# Autodesk Inventor assembly: tip_3_n_base_ass
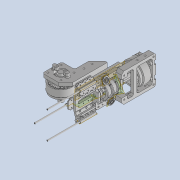
[picture p0: Inventor's stored thumbnail of the model, 180x180]
Saved by Autodesk Inventor 2020 (Build 240168000, 168)
## iProperties
Created: 2021-10-06
Part Number: tip_3_n_base_ass
Document SubType Name: Assembly
Designer: Shuang Peng
Author: Shuang Peng
## Documents named in this file (14)
- D:\projects-3\torque fb tip\hardware\tip_3\tip_3_n_base_ass.iam
- D:\projects-3\torque fb tip\hardware\tip_3\roller_n_1.ipt
- D:\projects-3\torque fb tip\hardware\tip_3\bearing_hh_1.ipt
- D:\projects-3\torque fb tip\hardware\tip_3\bearing_3_6_2.ipt
- D:\projects-3\torque fb tip\hardware\tip_3\pin3_40.ipt
- D:\projects-3\torque fb tip\hardware\tip_3\end_shell_n_1.ipt
- D:\projects-3\torque fb tip\hardware\tip_3\c_roller_1.ipt
- D:\projects-3\torque fb tip\hardware\tip_3\bl_tube_ass_2.iam
- D:\projects-3\torque fb tip\hardware\tip_3\ext_pin_shell_2.ipt
- D:\projects-3\torque fb tip\hardware\tip_3\mot_test_enc_hh_1.ipt
- D:\projects-3\torque fb tip\hardware\tip_3\mot_27_ass.iam
- D:\projects-3\torque fb tip\hardware\tip_3\mot_trans_1.ipt
- D:\projects-3\torque fb tip\hardware\tip_3\arc_wheel_shell_1.ipt
- D:\projects-3\torque fb tip\hardware\tip_3\tendon_wh_1_mod.ipt
## Components (24 placed, 13 different names)
1. roller_n_1:1 — Insert:1, Insert:2, Insert:5
2. roller_n_1:2 — Insert:1, Insert:2, Insert:6, Flush:3
3. bearing_hh_1:1 — Insert:3, Flush:1, Flush:2
4. bearing_hh_1:2 — Insert:4, Flush:1, Insert:8
5. bearing_3_6_2:1 — Insert:4, Insert:6
6. bearing_3_6_2:2 — Insert:3, Insert:5, Insert:7
7. pin3_40:1 — Insert:7
8. end_shell_n_1:1 — Flush:2, Insert:8, Flush:3, Insert:10, Insert:12, Flush:4, Mate:1, Flush:5, Insert:17
9. c_roller_1:1 — Insert:9
10. bearing_3_6_2:3 — Insert:9, Insert:10
11. c_roller_1:2
12. bearing_3_6_2:4 — Insert:12
13. bl_tube_ass_2:1 [sub-assembly] — Insert:22, Insert:23
14. bl_tube_ass_2:2 [sub-assembly] — Insert:20, Insert:21
15. bl_tube_ass_2:3 [sub-assembly] — Insert:18, Insert:19
16. ext_pin_shell_2:1 — Flush:4, Mate:1, Flush:5, Angle:1, Insert:18, Insert:19, Insert:20, Insert:21, Insert:22, Insert:23, Flush:6, Insert:24, Insert:25
17. mot_test_enc_hh_1:1 — Insert:13, Insert:14, Angle:1
18. mot_27_ass:1 [sub-assembly] — Insert:13, Insert:14, Insert:15, Insert:16
19. mot_trans_1:1 — Insert:15, Insert:16, Insert:17
20. arc_wheel_shell_1:1 — Flush:6, Insert:24, Insert:25, Insert:27, Flush:7
21. c_roller_1:3
22. bearing_3_6_2:5 — Insert:27
23. mot_27_ass:2 [sub-assembly] — Flush:7, Insert:28, Insert:29
24. tendon_wh_1_mod:1 — Insert:28, Insert:29
## Relationships (38: Insert 29, Flush 7, Mate 1, Angle 1)
- Insert:1: roller_n_1:1 ↔ roller_n_1:2
- Insert:2: roller_n_1:1 ↔ roller_n_1:2
- Insert:3: bearing_hh_1:1 ↔ bearing_3_6_2:2
- Insert:4: bearing_hh_1:2 ↔ bearing_3_6_2:1
- Insert:5: roller_n_1:1 ↔ bearing_3_6_2:2
- Insert:6 (0.3 mm): roller_n_1:2 ↔ bearing_3_6_2:1
- Flush:1: bearing_hh_1:1 ↔ bearing_hh_1:2
- Insert:7 (-3 mm): bearing_3_6_2:2 ↔ pin3_40:1
- Flush:2: bearing_hh_1:1 ↔ end_shell_n_1:1
- Insert:8: bearing_hh_1:2 ↔ end_shell_n_1:1
- Flush:3: roller_n_1:2 ↔ end_shell_n_1:1
- Insert:9: c_roller_1:1 ↔ bearing_3_6_2:3
- Insert:10: end_shell_n_1:1 ↔ bearing_3_6_2:3
- [Insert]: c_roller_1:2 ↔ bearing_3_6_2:4
- Insert:12: end_shell_n_1:1 ↔ bearing_3_6_2:4
- Flush:4 (1 mm): end_shell_n_1:1 ↔ ext_pin_shell_2:1
- Mate:1: end_shell_n_1:1 ↔ ext_pin_shell_2:1
- Flush:5 (6 mm): end_shell_n_1:1 ↔ ext_pin_shell_2:1
- Insert:13: mot_test_enc_hh_1:1 ↔ mot_27_ass:1
- Insert:14: mot_test_enc_hh_1:1 ↔ mot_27_ass:1
- Insert:15: mot_27_ass:1 ↔ mot_trans_1:1
- Insert:16: mot_27_ass:1 ↔ mot_trans_1:1
- Insert:17 (2 mm): end_shell_n_1:1 ↔ mot_trans_1:1
- Angle:1 (0 deg): ext_pin_shell_2:1 ↔ mot_test_enc_hh_1:1
- Insert:18: bl_tube_ass_2:3 ↔ ext_pin_shell_2:1
- Insert:19: bl_tube_ass_2:3 ↔ ext_pin_shell_2:1
- Insert:20: bl_tube_ass_2:2 ↔ ext_pin_shell_2:1
- Insert:21: bl_tube_ass_2:2 ↔ ext_pin_shell_2:1
- Insert:22: bl_tube_ass_2:1 ↔ ext_pin_shell_2:1
- Insert:23: bl_tube_ass_2:1 ↔ ext_pin_shell_2:1
- Flush:6: ext_pin_shell_2:1 ↔ arc_wheel_shell_1:1
- Insert:24: ext_pin_shell_2:1 ↔ arc_wheel_shell_1:1
- Insert:25: ext_pin_shell_2:1 ↔ arc_wheel_shell_1:1
- [Insert]: c_roller_1:3 ↔ bearing_3_6_2:5
- Insert:27: arc_wheel_shell_1:1 ↔ bearing_3_6_2:5
- Flush:7 (3 mm): arc_wheel_shell_1:1 ↔ mot_27_ass:2
- Insert:28: mot_27_ass:2 ↔ tendon_wh_1_mod:1
- Insert:29: mot_27_ass:2 ↔ tendon_wh_1_mod:1
## Named parameters: d13_d11 = 0 mm, d61_d13_d11 = 0 mm
